# Autodesk Inventor assembly: RT_FRM_V2_A_002_Dynamics
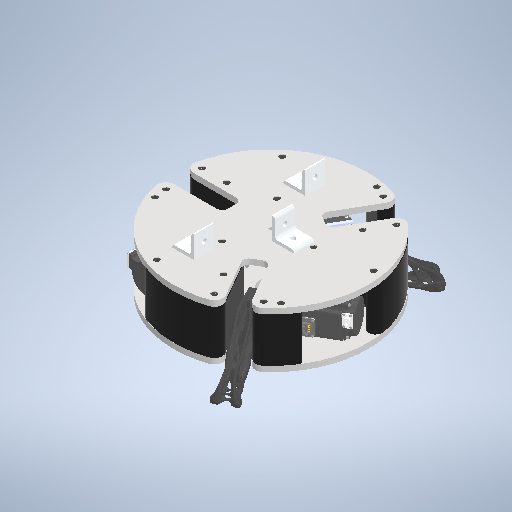
[picture p0: Inventor's stored thumbnail of the model, 512x512]
Saved by Autodesk Inventor 2025.3 (Build 293356000, 356)
## iProperties
Created: 2026-05-11
Part Number: RT_FRM_V2_A_002_Dynamics
Document SubType Name: Assembly
Designer: louis
Mass: 9176.21 g
Surface Area: 8073.41 cm^2
Volume: 2320.58 cm^3
Density: 3.95427 g/cm^3
Author: louis
## Documents named in this file (10)
- C:\Users\louis\OneDrive\Desktop\R_Trident\02_CAD\04_Subassemblies\RT_FRM_V2_A_002_Dynamics.iam
- C:\Users\louis\OneDrive\Desktop\R_Trident\02_CAD\03_Parts_Custom\RT_FRM_V2_MC_004_TopDynamicsPlate.ipt
- C:\Users\louis\OneDrive\Desktop\R_Trident\02_CAD\03_Parts_Custom\RT_FRM_V2_MC_004_BottomDynamicsPlate.ipt
- C:\Users\louis\OneDrive\Desktop\R_Trident\02_CAD\04_Subassemblies\RT_ARM_V2_A_001.iam
- C:\Users\louis\OneDrive\Desktop\R_Trident\02_CAD\03_Parts_Custom\RT_FRM_V2_MC_004_IntermediateB_DynamicsPlate.ipt
- C:\Users\louis\OneDrive\Desktop\R_Trident\02_CAD\03_Parts_Custom\RT_FRM_V2_MC_004_IntermediateDynamicsPlate.ipt
- C:\Users\louis\OneDrive\Documents\Inventor\Content Center Files\R2025\en-US\ISO 4762(2)\ISO 4762 - M5 x 30ISO.ipt
- C:\Users\louis\OneDrive\Documents\Inventor\Content Center Files\R2025\en-US\ISO 10642(1)\ISO 10642 - M5 x  20.ipt
- C:\Users\louis\OneDrive\Documents\Inventor\Content Center Files\R2025\en-US\ISO 4032(2)\ISO 4032 - M5 - ISO.ipt
- C:\Users\louis\OneDrive\Desktop\R_Trident\02_CAD\01_Standard_Parts\03_FRM_Fastener\4040L-ALU.ipt
## Components (71 placed, 9 different names)
1. RT_FRM_V2_MC_004_TopDynamicsPlate:1 — Flush:1, Flush:2, Flush:3, Flush:4, Flush:5, Mate:1, Mate:9, Mate:10, Mate:11, Mate:12, Mate:13, Mate:15, Mate:20, Mate:21, Mate:22, Mate:23, Mate:24, Mate:25, Mate:26, Mate:27, Mate:28, Mate:29, Mate:30, Mate:31, Mate:32, Mate:33, Mate:34, Mate:35, Mate:36, Mate:37, Mate:53, Mate:54, Mate:55, Mate:56, Mate:57, Mate:58
2. RT_FRM_V2_MC_004_BottomDynamicsPlate:1 — Flush:4, Flush:5, Mate:1, Mate:2, Mate:3, Mate:4, Mate:5, Mate:6, Mate:7, Mate:8, Mate:14, Mate:16, Mate:17, Mate:18, Mate:19, Insert:1, Insert:2, Insert:3, Insert:4, Insert:5, Insert:6, Insert:7, Insert:8, Insert:9, Insert:10, Insert:11, Insert:12, Mate:38, Mate:39, Mate:40, Mate:41, Mate:42, Mate:43, Mate:44, Mate:45, Mate:46, Mate:47, Mate:48, Mate:49, Mate:50, Mate:51, Mate:52
3. RT_ARM_V2_A_001:1 [sub-assembly] — Mate:6, Mate:7, Insert:21, Insert:22, Insert:23, Insert:24
4. RT_ARM_V2_A_001:2 [sub-assembly] — Mate:4, Mate:5, Insert:17, Insert:18, Insert:19, Insert:20
5. RT_ARM_V2_A_001:3 [sub-assembly] — Mate:2, Mate:3, Insert:13, Insert:14, Insert:15, Insert:16
6. RT_FRM_V2_MC_004_IntermediateB_DynamicsPlate:1 — Mate:8, Mate:9
7. RT_FRM_V2_MC_004_IntermediateB_DynamicsPlate:2 — Mate:12, Mate:13
8. RT_FRM_V2_MC_004_IntermediateB_DynamicsPlate:3 — Mate:10, Mate:11
9. RT_FRM_V2_MC_004_IntermediateDynamicsPlate:1 — Mate:14, Mate:15
10. RT_FRM_V2_MC_004_IntermediateDynamicsPlate:2 — Mate:16, Mate:17
11. RT_FRM_V2_MC_004_IntermediateDynamicsPlate:3 — Mate:18, Mate:19
12. ISO 4762 M5 x 30:1 — Insert:1
13. ISO 4762 M5 x 30:2 — Insert:2
14. ISO 4762 M5 x 30:3 — Insert:3
15. ISO 4762 M5 x 30:4 — Insert:4
16. ISO 4762 M5 x 30:5 — Insert:5
17. ISO 4762 M5 x 30:6 — Insert:6
18. ISO 4762 M5 x 30:7 — Insert:7
19. ISO 4762 M5 x 30:8 — Insert:8
20. ISO 4762 M5 x 30:9 — Insert:9
21. ISO 4762 M5 x 30:10 — Insert:10
22. ISO 4762 M5 x 30:11 — Insert:11
23. ISO 4762 M5 x 30:12 — Insert:12
24. ISO 10642 M5x20:1 — Mate:20
25. ISO 10642 M5x20:2 — Mate:21
26. ISO 10642 M5x20:3 — Mate:22
27. ISO 10642 M5x20:4 — Mate:23
28. ISO 10642 M5x20:5 — Mate:24
29. ISO 10642 M5x20:6 — Mate:25
30. ISO 10642 M5x20:7 — Mate:26
31. ISO 10642 M5x20:8 — Mate:27
32. ISO 10642 M5x20:9 — Mate:28
33. ISO 10642 M5x20:10 — Mate:29
34. ISO 10642 M5x20:11 — Mate:30
35. ISO 10642 M5x20:12 — Mate:31
36. ISO 10642 M5x20:13 — Mate:32
37. ISO 10642 M5x20:14 — Mate:33
38. ISO 10642 M5x20:15 — Mate:34
39. ISO 10642 M5x20:16 — Mate:35
40. ISO 10642 M5x20:17 — Mate:36
41. ISO 10642 M5x20:18 — Mate:37
42. ISO 10642 M5x20:19 — Mate:38
43. ISO 10642 M5x20:20 — Mate:39
44. ISO 10642 M5x20:21 — Mate:40
45. ISO 10642 M5x20:22 — Mate:41
46. ISO 10642 M5x20:23 — Mate:42
47. ISO 10642 M5x20:24 — Mate:43
48. ISO 10642 M5x20:25 — Mate:44
49. ISO 10642 M5x20:26 — Mate:45
50. ISO 10642 M5x20:27 — Mate:46
51. ISO 10642 M5x20:28 — Mate:47
52. ISO 10642 M5x20:29 — Mate:48
53. ISO 10642 M5x20:30 — Mate:49
54. ISO 10642 M5x20:31 — Mate:50
55. ISO 10642 M5x20:32 — Mate:51
56. ISO 10642 M5x20:33 — Mate:52
57. ISO 4032 M5:1 — Insert:13
58. ISO 4032 M5:2 — Insert:14
59. ISO 4032 M5:3 — Insert:15
60. ISO 4032 M5:4 — Insert:16
61. ISO 4032 M5:5 — Insert:17
62. ISO 4032 M5:6 — Insert:18
63. ISO 4032 M5:7 — Insert:19
64. ISO 4032 M5:8 — Insert:20
65. ISO 4032 M5:9 — Insert:21
66. ISO 4032 M5:10 — Insert:22
67. ISO 4032 M5:11 — Insert:23
68. ISO 4032 M5:12 — Insert:24
69. 4040L-ALU:1 — Mate:53, Mate:54, Flush:6, Mate:59
70. 4040L-ALU:2 — Mate:57, Mate:58, Flush:6
71. 4040L-ALU:3 — Mate:55, Mate:56, Mate:59
## Relationships (89: Mate 59, Insert 24, Flush 6)
- Flush:1: RT_FRM_V2_MC_004_TopDynamicsPlate:1
- Flush:2: RT_FRM_V2_MC_004_TopDynamicsPlate:1
- Flush:3: RT_FRM_V2_MC_004_TopDynamicsPlate:1
- Flush:4: RT_FRM_V2_MC_004_TopDynamicsPlate:1 ↔ RT_FRM_V2_MC_004_BottomDynamicsPlate:1
- Flush:5: RT_FRM_V2_MC_004_TopDynamicsPlate:1 ↔ RT_FRM_V2_MC_004_BottomDynamicsPlate:1
- Mate:1 (80 mm): RT_FRM_V2_MC_004_TopDynamicsPlate:1 ↔ RT_FRM_V2_MC_004_BottomDynamicsPlate:1
- Mate:2: RT_FRM_V2_MC_004_BottomDynamicsPlate:1 ↔ RT_ARM_V2_A_001:3
- Mate:3: RT_FRM_V2_MC_004_BottomDynamicsPlate:1 ↔ RT_ARM_V2_A_001:3
- Mate:4: RT_FRM_V2_MC_004_BottomDynamicsPlate:1 ↔ RT_ARM_V2_A_001:2
- Mate:5: RT_FRM_V2_MC_004_BottomDynamicsPlate:1 ↔ RT_ARM_V2_A_001:2
- Mate:6: RT_FRM_V2_MC_004_BottomDynamicsPlate:1 ↔ RT_ARM_V2_A_001:1
- Mate:7: RT_FRM_V2_MC_004_BottomDynamicsPlate:1 ↔ RT_ARM_V2_A_001:1
- Mate:8: RT_FRM_V2_MC_004_BottomDynamicsPlate:1 ↔ RT_FRM_V2_MC_004_IntermediateB_DynamicsPlate:1
- Mate:9: RT_FRM_V2_MC_004_TopDynamicsPlate:1 ↔ RT_FRM_V2_MC_004_IntermediateB_DynamicsPlate:1
- Mate:10: RT_FRM_V2_MC_004_TopDynamicsPlate:1 ↔ RT_FRM_V2_MC_004_IntermediateB_DynamicsPlate:3
- Mate:11: RT_FRM_V2_MC_004_TopDynamicsPlate:1 ↔ RT_FRM_V2_MC_004_IntermediateB_DynamicsPlate:3
- Mate:12: RT_FRM_V2_MC_004_TopDynamicsPlate:1 ↔ RT_FRM_V2_MC_004_IntermediateB_DynamicsPlate:2
- Mate:13: RT_FRM_V2_MC_004_TopDynamicsPlate:1 ↔ RT_FRM_V2_MC_004_IntermediateB_DynamicsPlate:2
- Mate:14: RT_FRM_V2_MC_004_BottomDynamicsPlate:1 ↔ RT_FRM_V2_MC_004_IntermediateDynamicsPlate:1
- Mate:15: RT_FRM_V2_MC_004_TopDynamicsPlate:1 ↔ RT_FRM_V2_MC_004_IntermediateDynamicsPlate:1
- Mate:16: RT_FRM_V2_MC_004_BottomDynamicsPlate:1 ↔ RT_FRM_V2_MC_004_IntermediateDynamicsPlate:2
- Mate:17: RT_FRM_V2_MC_004_BottomDynamicsPlate:1 ↔ RT_FRM_V2_MC_004_IntermediateDynamicsPlate:2
- Mate:18: RT_FRM_V2_MC_004_BottomDynamicsPlate:1 ↔ RT_FRM_V2_MC_004_IntermediateDynamicsPlate:3
- Mate:19: RT_FRM_V2_MC_004_BottomDynamicsPlate:1 ↔ RT_FRM_V2_MC_004_IntermediateDynamicsPlate:3
- Insert:1: RT_FRM_V2_MC_004_BottomDynamicsPlate:1 ↔ ISO 4762 M5 x 30:1
- Insert:2: RT_FRM_V2_MC_004_BottomDynamicsPlate:1 ↔ ISO 4762 M5 x 30:2
- Insert:3: RT_FRM_V2_MC_004_BottomDynamicsPlate:1 ↔ ISO 4762 M5 x 30:3
- Insert:4: RT_FRM_V2_MC_004_BottomDynamicsPlate:1 ↔ ISO 4762 M5 x 30:4
- Insert:5: RT_FRM_V2_MC_004_BottomDynamicsPlate:1 ↔ ISO 4762 M5 x 30:5
- Insert:6: RT_FRM_V2_MC_004_BottomDynamicsPlate:1 ↔ ISO 4762 M5 x 30:6
- Insert:7: RT_FRM_V2_MC_004_BottomDynamicsPlate:1 ↔ ISO 4762 M5 x 30:7
- Insert:8: RT_FRM_V2_MC_004_BottomDynamicsPlate:1 ↔ ISO 4762 M5 x 30:8
- Insert:9: RT_FRM_V2_MC_004_BottomDynamicsPlate:1 ↔ ISO 4762 M5 x 30:9
- Insert:10: RT_FRM_V2_MC_004_BottomDynamicsPlate:1 ↔ ISO 4762 M5 x 30:10
- Insert:11: RT_FRM_V2_MC_004_BottomDynamicsPlate:1 ↔ ISO 4762 M5 x 30:11
- Insert:12: RT_FRM_V2_MC_004_BottomDynamicsPlate:1 ↔ ISO 4762 M5 x 30:12
- Mate:20: RT_FRM_V2_MC_004_TopDynamicsPlate:1 ↔ ISO 10642 M5x20:1
- Mate:21: RT_FRM_V2_MC_004_TopDynamicsPlate:1 ↔ ISO 10642 M5x20:2
- Mate:22: RT_FRM_V2_MC_004_TopDynamicsPlate:1 ↔ ISO 10642 M5x20:3
- Mate:23: RT_FRM_V2_MC_004_TopDynamicsPlate:1 ↔ ISO 10642 M5x20:4
- Mate:24: RT_FRM_V2_MC_004_TopDynamicsPlate:1 ↔ ISO 10642 M5x20:5
- Mate:25: RT_FRM_V2_MC_004_TopDynamicsPlate:1 ↔ ISO 10642 M5x20:6
- Mate:26: RT_FRM_V2_MC_004_TopDynamicsPlate:1 ↔ ISO 10642 M5x20:7
- Mate:27: RT_FRM_V2_MC_004_TopDynamicsPlate:1 ↔ ISO 10642 M5x20:8
- Mate:28: RT_FRM_V2_MC_004_TopDynamicsPlate:1 ↔ ISO 10642 M5x20:9
- Mate:29: RT_FRM_V2_MC_004_TopDynamicsPlate:1 ↔ ISO 10642 M5x20:10
- Mate:30: RT_FRM_V2_MC_004_TopDynamicsPlate:1 ↔ ISO 10642 M5x20:11
- Mate:31: RT_FRM_V2_MC_004_TopDynamicsPlate:1 ↔ ISO 10642 M5x20:12
- Mate:32: RT_FRM_V2_MC_004_TopDynamicsPlate:1 ↔ ISO 10642 M5x20:13
- Mate:33: RT_FRM_V2_MC_004_TopDynamicsPlate:1 ↔ ISO 10642 M5x20:14
- Mate:34: RT_FRM_V2_MC_004_TopDynamicsPlate:1 ↔ ISO 10642 M5x20:15
- Mate:35: RT_FRM_V2_MC_004_TopDynamicsPlate:1 ↔ ISO 10642 M5x20:16
- Mate:36: RT_FRM_V2_MC_004_TopDynamicsPlate:1 ↔ ISO 10642 M5x20:17
- Mate:37: RT_FRM_V2_MC_004_TopDynamicsPlate:1 ↔ ISO 10642 M5x20:18
- Mate:38: RT_FRM_V2_MC_004_BottomDynamicsPlate:1 ↔ ISO 10642 M5x20:19
- Mate:39: RT_FRM_V2_MC_004_BottomDynamicsPlate:1 ↔ ISO 10642 M5x20:20
- Mate:40: RT_FRM_V2_MC_004_BottomDynamicsPlate:1 ↔ ISO 10642 M5x20:21
- Mate:41: RT_FRM_V2_MC_004_BottomDynamicsPlate:1 ↔ ISO 10642 M5x20:22
- Mate:42: RT_FRM_V2_MC_004_BottomDynamicsPlate:1 ↔ ISO 10642 M5x20:23
- Mate:43: RT_FRM_V2_MC_004_BottomDynamicsPlate:1 ↔ ISO 10642 M5x20:24
- Mate:44: RT_FRM_V2_MC_004_BottomDynamicsPlate:1 ↔ ISO 10642 M5x20:25
- Mate:45: RT_FRM_V2_MC_004_BottomDynamicsPlate:1 ↔ ISO 10642 M5x20:26
- Mate:46: RT_FRM_V2_MC_004_BottomDynamicsPlate:1 ↔ ISO 10642 M5x20:27
- Mate:47: RT_FRM_V2_MC_004_BottomDynamicsPlate:1 ↔ ISO 10642 M5x20:28
- Mate:48: RT_FRM_V2_MC_004_BottomDynamicsPlate:1 ↔ ISO 10642 M5x20:29
- Mate:49: RT_FRM_V2_MC_004_BottomDynamicsPlate:1 ↔ ISO 10642 M5x20:30
- Mate:50: RT_FRM_V2_MC_004_BottomDynamicsPlate:1 ↔ ISO 10642 M5x20:31
- Mate:51: RT_FRM_V2_MC_004_BottomDynamicsPlate:1 ↔ ISO 10642 M5x20:32
- Mate:52: RT_FRM_V2_MC_004_BottomDynamicsPlate:1 ↔ ISO 10642 M5x20:33
- Insert:13: RT_ARM_V2_A_001:3 ↔ ISO 4032 M5:1
- Insert:14: RT_ARM_V2_A_001:3 ↔ ISO 4032 M5:2
- Insert:15: RT_ARM_V2_A_001:3 ↔ ISO 4032 M5:3
- Insert:16: RT_ARM_V2_A_001:3 ↔ ISO 4032 M5:4
- Insert:17: RT_ARM_V2_A_001:2 ↔ ISO 4032 M5:5
- Insert:18: RT_ARM_V2_A_001:2 ↔ ISO 4032 M5:6
- Insert:19: RT_ARM_V2_A_001:2 ↔ ISO 4032 M5:7
- Insert:20: RT_ARM_V2_A_001:2 ↔ ISO 4032 M5:8
- Insert:21: RT_ARM_V2_A_001:1 ↔ ISO 4032 M5:9
- Insert:22: RT_ARM_V2_A_001:1 ↔ ISO 4032 M5:10
- Insert:23: RT_ARM_V2_A_001:1 ↔ ISO 4032 M5:11
- Insert:24: RT_ARM_V2_A_001:1 ↔ ISO 4032 M5:12
- Mate:53: RT_FRM_V2_MC_004_TopDynamicsPlate:1 ↔ 4040L-ALU:1
- Mate:54: RT_FRM_V2_MC_004_TopDynamicsPlate:1 ↔ 4040L-ALU:1
- Mate:55: RT_FRM_V2_MC_004_TopDynamicsPlate:1 ↔ 4040L-ALU:3
- Mate:56: RT_FRM_V2_MC_004_TopDynamicsPlate:1 ↔ 4040L-ALU:3
- Mate:57: RT_FRM_V2_MC_004_TopDynamicsPlate:1 ↔ 4040L-ALU:2
- Mate:58: RT_FRM_V2_MC_004_TopDynamicsPlate:1 ↔ 4040L-ALU:2
- Flush:6: 4040L-ALU:1 ↔ 4040L-ALU:2
- Mate:59: 4040L-ALU:1 ↔ 4040L-ALU:3
